# Autodesk Inventor assembly: robot
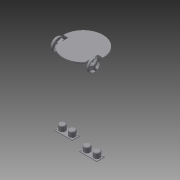
[picture p0: Inventor's stored thumbnail of the model, 180x180]
Saved by Autodesk Inventor 2015 (Build 190159000, 159)
## iProperties
Created: 2014-10-25
Part Number: robot
Document SubType Name: Assembly
Designer: Colin
Author: Colin
## Documents named in this file (4)
- E:\Users\Colin\Documents\college\marc\MicroMouse\robot.iam
- E:\Users\Colin\Documents\college\marc\MicroMouse\base.ipt
- E:\Users\Colin\Documents\college\marc\MicroMouse\wheel_assembly.iam
- E:\Users\Colin\Documents\college\marc\MicroMouse\ping.ipt
## Components (5 placed, 3 different names)
1. base:1 — Flush:1, Flush:2, Mate:5, Mate:7, Mate:8
2. wheel_assembly:1 [sub-assembly] — Flush:1, Mate:5
3. wheel_assembly:2 [sub-assembly] — Flush:2, Mate:7, Mate:8
4. ping:1
5. ping:2
## Relationships (5: Mate 3, Flush 2)
- Flush:1: base:1 ↔ wheel_assembly:1
- Flush:2: base:1 ↔ wheel_assembly:2
- Mate:5: base:1 ↔ wheel_assembly:1
- Mate:7: base:1 ↔ wheel_assembly:2
- Mate:8: base:1 ↔ wheel_assembly:2
